# Autodesk Inventor assembly: Ball Picker Upper
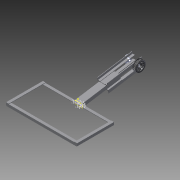
[picture p0: Inventor's stored thumbnail of the model, 180x180]
Saved by Autodesk Inventor 2015 (Build 190159000, 159)
## iProperties
Created: 2016-02-06
Part Number: Ball Picker Upper
Document SubType Name: Assembly
Designer: sethbattis
Author: sethbattis
## Documents named in this file (6)
- \\area51\team3566\cad\FRC 2016\Ball Picker Upper.iam
- \\area51\team3566\cad\FRC 2016\Prow rev2.ipt
- \\area51\team3566\cad\FRC 2016\Imported Components\42 tooth HTD Pulley half 2014.ipt\42 tooth HTD Pulley half 2014.ipt.ipt
- \\area51\team3566\cad\FRC 2016\Imported Components\500EX Hex Hub.ipt\500EX Hex Hub.ipt.ipt
- 42 tooth HTD Pulley half 2014.ipt
- 500EX Hex Hub.ipt
## Components (5 placed, 3 different names)
1. Prow rev2:1 — Mate:7, Mate:8
2. 42 tooth HTD Pulley half 2014.ipt:1 — Mate:1, Mate:2, Mate:3
3. 42 tooth HTD Pulley half 2014.ipt:2 — Mate:1, Mate:2, Mate:3, Mate:4, Mate:5, Mate:6
4. 500EX Hex Hub.ipt:1 — Mate:4, Mate:5, Mate:6, Mate:7, Mate:9, Mate:10
5. 500EX Hex Hub.ipt:2 — Mate:8, Mate:9, Mate:10
## Relationships (10: Mate 10)
- Mate:1: 42 tooth HTD Pulley half 2014.ipt:1 ↔ 42 tooth HTD Pulley half 2014.ipt:2
- Mate:2: 42 tooth HTD Pulley half 2014.ipt:1 ↔ 42 tooth HTD Pulley half 2014.ipt:2
- Mate:3: 42 tooth HTD Pulley half 2014.ipt:1 ↔ 42 tooth HTD Pulley half 2014.ipt:2
- Mate:4: 42 tooth HTD Pulley half 2014.ipt:2 ↔ 500EX Hex Hub.ipt:1
- Mate:5: 42 tooth HTD Pulley half 2014.ipt:2 ↔ 500EX Hex Hub.ipt:1
- Mate:6: 42 tooth HTD Pulley half 2014.ipt:2 ↔ 500EX Hex Hub.ipt:1
- Mate:7: Prow rev2:1 ↔ 500EX Hex Hub.ipt:1
- Mate:8: Prow rev2:1 ↔ 500EX Hex Hub.ipt:2
- Mate:9: 500EX Hex Hub.ipt:1 ↔ 500EX Hex Hub.ipt:2
- Mate:10: 500EX Hex Hub.ipt:1 ↔ 500EX Hex Hub.ipt:2
